# Autodesk Inventor assembly: full assembly
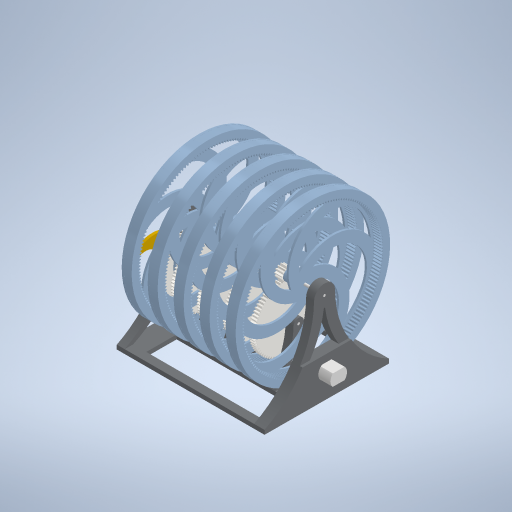
[picture p0: Inventor's stored thumbnail of the model, 512x512]
Saved by Autodesk Inventor 2023 (Build 270158000, 158)
## iProperties
Created: 2023-03-30
Part Number: full assembly
Document SubType Name: Assembly
Designer: dverd
Author: dverd
## Documents named in this file (12)
- C:\Users\AggyT\Desktop\College\Undergraduate Archives\Year 3\Spring 2023\ME354\Lab\Final Project\CAD\CAD\full assembly.iam
- C:\Users\AggyT\Desktop\College\Undergraduate Archives\Year 3\Spring 2023\ME354\Lab\Final Project\CAD\CAD\main rod.ipt
- C:\Users\AggyT\Desktop\College\Undergraduate Archives\Year 3\Spring 2023\ME354\Lab\Final Project\CAD\CAD\driven gear(1).ipt
- C:\Users\AggyT\Desktop\College\Undergraduate Archives\Year 3\Spring 2023\ME354\Lab\Final Project\CAD\CAD\repeated section(4).iam
- C:\Users\AggyT\Desktop\College\Undergraduate Archives\Year 3\Spring 2023\ME354\Lab\Final Project\CAD\CAD\end section(1).iam
- C:\Users\AggyT\Desktop\College\Undergraduate Archives\Year 3\Spring 2023\ME354\Lab\Final Project\CAD\CAD\tranfer gear(4).ipt
- C:\Users\AggyT\Desktop\College\Undergraduate Archives\Year 3\Spring 2023\ME354\Lab\Final Project\CAD\CAD\tranfer gear end(1).ipt
- C:\Users\AggyT\Desktop\College\Undergraduate Archives\Year 3\Spring 2023\ME354\Lab\Final Project\CAD\CAD\fan.ipt
- C:\Users\AggyT\Desktop\College\Undergraduate Archives\Year 3\Spring 2023\ME354\Lab\Final Project\CAD\CAD\motor 12v.ipt
- C:\Users\AggyT\Desktop\College\Undergraduate Archives\Year 3\Spring 2023\ME354\Lab\Final Project\CAD\CAD\transfer gear rod.ipt
- C:\Users\AggyT\Desktop\College\Undergraduate Archives\Year 3\Spring 2023\ME354\Lab\Final Project\CAD\CAD\transfer gear rod end.ipt
- C:\Users\AggyT\Desktop\College\Undergraduate Archives\Year 3\Spring 2023\ME354\Lab\Final Project\CAD\CAD\base assembly(1).iam
## Components (20 placed, 10 different names)
1. main rod:1 — Mate:17, Mate:19, Mate:36, Flush:20
2. Spur Gear1:1 — Flush:6
3. repeated section(4):1 [sub-assembly] — Mate:13, Mate:14, Mate:16, Flush:12
4. repeated section(4):2 [sub-assembly] — Mate:11, Mate:12, Mate:14, Mate:20
5. repeated section(4):3 [sub-assembly] — Mate:12, Mate:13, Mate:15, Mate:16, Mate:17, Flush:6
6. repeated section(4):4 [sub-assembly] — Mate:11, Mate:15
7. end section(1):1 [sub-assembly] — Mate:19, Mate:20, Flush:13
8. Spur Gear2:1 — Mate:21, Mate:22, Mate:23, Flush:9, Flush:10, Flush:23
9. Spur Gear2:2 — Mate:21, Flush:9, Flush:11
10. Spur Gear2:3 — Mate:22, Flush:11, Mate:26
11. Spur Gear2:4 — Mate:23, Flush:10, Flush:12, Mate:38
12. Spur Gear2:5 — Mate:26, Flush:13, Flush:24
13. fan:1 — Mate:35, Flush:19
14. motor 12v:1 — Mate:39, Angle:1, Flush:21
15. transfer gear rod:1 — Mate:31, Mate:32, Flush:17, Mate:37, Mate:38
16. transfer gear rod:2 — Mate:33, Flush:15, Flush:16
17. transfer gear rod:3 — Mate:31, Mate:33, Flush:15, Flush:22
18. transfer gear rod:4 — Mate:32, Flush:16, Flush:17, Flush:23
19. transfer gear rod end:1 — Mate:35, Flush:19, Mate:40, Flush:24
20. base assembly(1):1 [sub-assembly] — Mate:36, Flush:20, Mate:37, Mate:39, Angle:1, Flush:21, Flush:22, Mate:40
## Relationships (38: Mate 22, Flush 15, Angle 1)
- Mate:11: repeated section(4):2 ↔ repeated section(4):4
- Mate:12: repeated section(4):2 ↔ repeated section(4):3
- Mate:13: repeated section(4):1 ↔ repeated section(4):3
- Mate:14 (33.02 mm): repeated section(4):1 ↔ repeated section(4):2
- Mate:15 (33.02 mm): repeated section(4):3 ↔ repeated section(4):4
- Mate:16 (1.5875 mm): repeated section(4):1 ↔ repeated section(4):3
- Mate:17: main rod:1 ↔ repeated section(4):3
- Flush:6: Spur Gear1:1 ↔ repeated section(4):3
- Mate:19: main rod:1 ↔ end section(1):1
- Mate:20 (1.5875 mm): repeated section(4):2 ↔ end section(1):1
- Mate:21: Spur Gear2:1 ↔ Spur Gear2:2
- Mate:22: Spur Gear2:1 ↔ Spur Gear2:3
- Mate:23: Spur Gear2:1 ↔ Spur Gear2:4
- Flush:9 (31.4452 mm): Spur Gear2:1 ↔ Spur Gear2:2
- Flush:10 (31.4452 mm): Spur Gear2:1 ↔ Spur Gear2:4
- Flush:11 (31.4452 mm): Spur Gear2:2 ↔ Spur Gear2:3
- Flush:12: repeated section(4):1 ↔ Spur Gear2:4
- Mate:26: Spur Gear2:3 ↔ Spur Gear2:5
- Flush:13: end section(1):1 ↔ Spur Gear2:5
- Mate:31: transfer gear rod:1 ↔ transfer gear rod:3
- Mate:32: transfer gear rod:1 ↔ transfer gear rod:4
- Mate:33: transfer gear rod:2 ↔ transfer gear rod:3
- Flush:15 (31.4452 mm): transfer gear rod:2 ↔ transfer gear rod:3
- Flush:16 (31.4452 mm): transfer gear rod:2 ↔ transfer gear rod:4
- Flush:17 (31.4452 mm): transfer gear rod:1 ↔ transfer gear rod:4
- Mate:35: fan:1 ↔ transfer gear rod end:1
- Flush:19: fan:1 ↔ transfer gear rod end:1
- Mate:36: main rod:1 ↔ base assembly(1):1
- Flush:20: main rod:1 ↔ base assembly(1):1
- Mate:37: transfer gear rod:1 ↔ base assembly(1):1
- Mate:38: Spur Gear2:4 ↔ transfer gear rod:1
- Mate:39: motor 12v:1 ↔ base assembly(1):1
- Angle:1 (0 deg): motor 12v:1 ↔ base assembly(1):1
- Flush:21: motor 12v:1 ↔ base assembly(1):1
- Flush:22: transfer gear rod:3 ↔ base assembly(1):1
- Flush:23: Spur Gear2:1 ↔ transfer gear rod:4
- Mate:40: transfer gear rod end:1 ↔ base assembly(1):1
- Flush:24: Spur Gear2:5 ↔ transfer gear rod end:1
